# Autodesk Inventor assembly: Drivebase
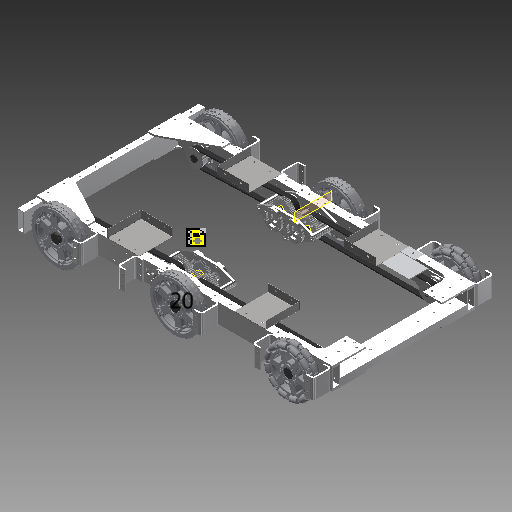
[picture p0: Inventor's stored thumbnail of the model, 512x512]
Saved by Autodesk Inventor 2019.4 (Build 234330000, 330)
## iProperties
Created: 2020-01-05
Part Number: Drivebase
Document SubType Name: Assembly
Designer: Mark
Mass: 13329.8 g
Surface Area: 29632.2 cm^2
Volume: 5059.07 cm^3
Density: 2.63483 g/cm^3
Author: Mark
## Documents named in this file (38)
- C:\Users\admin\Desktop\FRC 2020 Engineering\GitHub\7738-2020\CAD\Drivebase.iam
- C:\Users\admin\Desktop\FRC 2020 Engineering\GitHub\7738-2020\CAD\Main Extrusion.ipt
- C:\Users\admin\Desktop\FRC 2020 Engineering\GitHub\7738-2020\CAD\Back Extrusion.ipt
- C:\Users\admin\Desktop\FRC 2020 Engineering\GitHub\7738-2020\CAD\Bearing Block Assembly.iam
- C:\Users\admin\Desktop\FRC 2020 Engineering\GitHub\7738-2020\CAD\Gearbox\Drivebox.iam
- C:\Users\admin\Desktop\FRC 2020 Engineering\GitHub\7738-2020\CAD\End Extrusion.ipt
- C:\Users\admin\Desktop\FRC 2020 Engineering\GitHub\7738-2020\CAD\Gearbox\HTD 5M 30 20mm ID Keyed.ipt
- C:\Users\admin\Desktop\FRC 2020 Engineering\GitHub\7738-2020\CAD\Gearbox\30-30-870-HTD5M.ipt
- C:\Users\admin\Desktop\FRC 2020 Engineering\GitHub\7738-2020\CAD\Gearbox\30-30-750-HTD5M.ipt
- C:\Users\admin\Desktop\FRC 2020 Engineering\GitHub\7738-2020\CAD\Frontal Sheet Metal Support.ipt
- C:\Users\admin\Desktop\FRC 2020 Engineering\GitHub\7738-2020\CAD\Shaft-Secondary.ipt
- C:\Users\admin\Desktop\FRC 2020 Engineering\GitHub\7738-2020\CAD\Drivebase\Design Accelerator\Key Connection1.iam
- C:\Users\admin\Desktop\FRC 2020 Engineering\GitHub\7738-2020\CAD\Shaft-2.ipt
- C:\Users\admin\Desktop\FRC 2020 Engineering\GitHub\7738-2020\CAD\Back Brace.ipt
- C:\Users\admin\Desktop\FRC 2020 Engineering\GitHub\7738-2020\CAD\Back brace 2.ipt
- C:\Users\admin\Desktop\FRC 2020 Engineering\GitHub\7738-2020\CAD\Front Brace 2.ipt
- C:\Users\admin\Desktop\FRC 2020 Engineering\GitHub\7738-2020\CAD\Gearbox Support Thing.ipt
- C:\Users\admin\Desktop\FRC 2020 Engineering\GitHub\7738-2020\CAD\Main Extrusion_MIR.ipt
- C:\Users\admin\Desktop\FRC 2020 Engineering\GitHub\7738-2020\CAD\Bearing Block Assembly_MIR.iam
- C:\Users\admin\Desktop\FRC 2020 Engineering\GitHub\7738-2020\CAD\Gearbox\Drivebox_MIR.iam
- C:\Users\admin\Desktop\FRC 2020 Engineering\GitHub\7738-2020\CAD\Gearbox\HTD 5M 30 20mm ID Keyed_MIR.ipt
- C:\Users\admin\Desktop\FRC 2020 Engineering\GitHub\7738-2020\CAD\Gearbox\30-30-870-HTD5M_MIR.ipt
- C:\Users\admin\Desktop\FRC 2020 Engineering\GitHub\7738-2020\CAD\Gearbox\30-30-750-HTD5M_MIR.ipt
- C:\Users\admin\Desktop\FRC 2020 Engineering\GitHub\7738-2020\CAD\Frontal Sheet Metal Support_MIR.ipt
- C:\Users\admin\Desktop\FRC 2020 Engineering\GitHub\7738-2020\CAD\Shaft-Secondary_MIR.ipt
- C:\Users\admin\Desktop\FRC 2020 Engineering\GitHub\7738-2020\CAD\Drivebase\Design Accelerator\Key Connection1_MIR.iam
- C:\Users\admin\Desktop\FRC 2020 Engineering\GitHub\7738-2020\CAD\Shaft-Main_MIR.ipt
- C:\Users\admin\Desktop\FRC 2020 Engineering\GitHub\7738-2020\CAD\Shaft-2_MIR.ipt
- C:\Users\admin\Desktop\FRC 2020 Engineering\GitHub\7738-2020\CAD\Back Brace_MIR.ipt
- C:\Users\admin\Desktop\FRC 2020 Engineering\GitHub\7738-2020\CAD\Back brace 2_MIR.ipt
- C:\Users\admin\Desktop\FRC 2020 Engineering\GitHub\7738-2020\CAD\Gearbox Support Thing_MIR.ipt
- C:\Users\admin\Desktop\FRC 2020 Engineering\GitHub\7738-2020\CAD\Shaft-Main.ipt
- C:\Users\admin\Desktop\FRC 2020 Engineering\GitHub\7738-2020\CAD\6_Omni-Directional_Wheel_217-2585.ipt
- C:\Users\admin\Desktop\FRC 2020 Engineering\GitHub\7738-2020\CAD\6_Traction_Wheel_-_1_Wide_217-2589.ipt
- C:\Users\admin\Desktop\FRC 2020 Engineering\GitHub\7738-2020\CAD\6_Traction_Tire_-_0_5_Wide_217-2860.ipt
- C:\Users\admin\Desktop\FRC 2020 Engineering\GitHub\7738-2020\CAD\Sheet Metal Support.ipt
- C:\Users\admin\Desktop\FRC 2020 Engineering\GitHub\7738-2020\CAD\Sheet Metal Support_MIR.ipt
- C:\Users\admin\Desktop\FRC 2020 Engineering\GitHub\7738-2020\Battery Support.ipt
## Components (75 placed, 37 different names)
1. Main Extrusion:1 — Mate:1, Flush:1, Flush:2, Mate:2, Mate:3, Mate:4, Mate:5, Mate:6, Mate:7, Mate:8, Mate:9, Mate:10, Mate:11, Mate:12, Mate:13, Mate:14, Mate:15, Mate:16, Mate:17, Mate:18, Mate:19, Mate:27, Mate:30, Flush:3, Mate:31, Flush:4, Flush:5, Flush:6, Flush:7, Mate:42, Mate:43, Flush:8, Mate:49, Flush:11, Mate:61, Flush:14, Flush:15, Mate:63, Flush:18, Flush:19, Mate:64, Flush:20, Flush:21, Mate:65, Flush:22, Mate:124, Flush:43, Flush:44, Mate:163, Mate:164, Mate:165, Mate:168, Mate:176, Mate:177, Mate:178, Mate:179, Mate:180, Mate:181
2. Back Extrusion:1 — Mate:1, Flush:1, Flush:2, Mate:50, Mate:119, Flush:39, Flush:40
3. Bearing Block Assembly:1 [sub-assembly] — Mate:2, Mate:3, Mate:4, Mate:32, Mate:33
4. Bearing Block Assembly:2 [sub-assembly] — Mate:5, Mate:6, Mate:7, Mate:34, Mate:35
5. Bearing Block Assembly:3 [sub-assembly] — Mate:11, Mate:12, Mate:13, Mate:53, Mate:127
6. Bearing Block Assembly:4 [sub-assembly] — Mate:8, Mate:9, Mate:10, Mate:126
7. Bearing Block Assembly:5 [sub-assembly] — Mate:14, Mate:15, Mate:16, Mate:60, Flush:13
8. Bearing Block Assembly:6 [sub-assembly] — Mate:17, Mate:18, Mate:19, Mate:37, Mate:132, Mate:133
9. Drivebox:1 [sub-assembly] — Mate:27, Mate:31, Flush:4, Mate:40, Mate:121
10. End Extrusion:1 — Mate:30, Flush:3, Flush:5, Flush:46
11. HTD 5M 30 20mm ID Keyed:1 — Mate:32, Mate:33, Mate:39, Mate:41
12. HTD 5M 30 20mm ID Keyed:2 — Mate:34, Mate:35, Mate:36, Mate:38
13. 30-30-870-HTD5M:1 — Mate:36, Mate:37, Mate:38
14. 30-30-730-HTD5M:1 — Mate:39, Mate:40, Mate:41
15. Frontal Sheet Metal Support:1 — Flush:6, Flush:7, Mate:42, Mate:44
16. Frontal Sheet Metal Support:2 — Mate:43, Flush:8, Mate:44
17. Frontal Sheet Metal Support:5 — Mate:49, Flush:11, Mate:50
18. Shaft-Secondary:1 — Mate:53, Mate:127, Mate:140, Mate:141
19. Shaft-Secondary:2 — Mate:126, Mate:134, Mate:135
20. Key Connection:1 [sub-assembly]
21. Shaft-2:1 — Mate:60, Flush:13
22. Back Brace:1 — Mate:61, Flush:14, Flush:15
23. Back brace 2:1 — Mate:63, Flush:18, Flush:19
24. Front Brace 2:1 — Mate:64, Flush:20, Flush:21
25. Gearbox Support Thing:1 — Mate:65, Flush:22, Mate:121
26. Main Extrusion_MIR:1 — Mate:66, Mate:67, Mate:68, Mate:69, Mate:70, Mate:71, Mate:72, Mate:73, Mate:74, Mate:75, Mate:76, Mate:77, Mate:78, Mate:79, Mate:80, Mate:81, Mate:82, Mate:83, Flush:23, Mate:89, Mate:90, Mate:101, Flush:24, Flush:25, Flush:26, Mate:103, Flush:27, Mate:104, Flush:30, Flush:31, Mate:114, Flush:34, Flush:35, Mate:116, Flush:38, Mate:118, Mate:119, Flush:39, Flush:40, Mate:122, Mate:123, Flush:41, Flush:42, Mate:125, Flush:45, Flush:56, Mate:166, Mate:167, Mate:169, Flush:61, Mate:170, Mate:171, Mate:172, Mate:173, Mate:174, Mate:175, Mate:182, Mate:183
27. Bearing Block Assembly_MIR:1 [sub-assembly] — Mate:66, Mate:67, Mate:68, Mate:91, Mate:92
28. Bearing Block Assembly_MIR:2 [sub-assembly] — Mate:69, Mate:70, Mate:71, Mate:93, Mate:94
29. Bearing Block Assembly_MIR:3 [sub-assembly] — Mate:72, Mate:73, Mate:74, Mate:107, Mate:129
30. Bearing Block Assembly_MIR:4 [sub-assembly] — Mate:75, Mate:76, Mate:77, Mate:128, Mate:130
31. Bearing Block Assembly_MIR:5 [sub-assembly] — Mate:78, Mate:79, Mate:80, Flush:29, Mate:113
32. Bearing Block Assembly_MIR:6 [sub-assembly] — Mate:81, Mate:82, Mate:83, Mate:96, Mate:110, Mate:145
33. Drivebox_MIR:1 [sub-assembly] — Flush:23, Mate:89, Mate:90, Mate:99, Mate:131
34. HTD 5M 30 20mm ID Keyed_MIR:1 — Mate:91, Mate:92, Mate:98, Mate:100
35. HTD 5M 30 20mm ID Keyed_MIR:2 — Mate:93, Mate:94, Mate:95, Mate:97
36. 30-30-870-HTD5M_MIR:1 — Mate:95, Mate:96, Mate:97
37. 30-30-730-HTD5M_MIR:1 — Mate:98, Mate:99, Mate:100
38. Frontal Sheet Metal Support_MIR:1 — Mate:101, Flush:24, Flush:25, Mate:102
39. Frontal Sheet Metal Support_MIR:2 — Mate:102, Flush:26, Mate:103
40. Frontal Sheet Metal Support_MIR:3 — Flush:27, Mate:104, Mate:122
41. Shaft-Secondary_MIR:1 — Mate:107, Mate:129, Mate:142, Mate:143
42. Shaft-Secondary_MIR:2 — Mate:128, Mate:130, Mate:136, Mate:137
43. Key Connection1_MIR:1 [sub-assembly]
44. Shaft-Main_MIR:1 — Mate:110, Mate:144, Mate:145, Mate:146
45. Shaft-2_MIR:1 — Flush:29, Mate:113
46. Back Brace_MIR:1 — Flush:30, Flush:31, Mate:114
47. Back brace 2_MIR:1 — Flush:34, Flush:35, Mate:116
48. Gearbox Support Thing_MIR:1 — Flush:38, Mate:118, Mate:131
49. Front Brace 2:2 — Mate:123, Flush:41, Flush:42, Mate:184
50. Front Brace 2:3 — Mate:124, Flush:43, Flush:44
51. Front Brace 2:4 — Mate:125, Flush:45, Flush:46
52. Shaft-Main:1 — Mate:132, Mate:133, Mate:138, Mate:139
53. 6_Omni-Directional_Wheel_217-2585:1 — Mate:136, Mate:137
54. 6_Omni-Directional_Wheel_217-2585:2 — Mate:134, Mate:135
55. 6_Traction_Wheel_-_1_Wide_217-2589:1 — Mate:144, Mate:146, Mate:159, Mate:160, Mate:161
56. 6_Traction_Wheel_-_1_Wide_217-2589:2 — Mate:140, Mate:141, Mate:147, Mate:148, Mate:149, Mate:150
57. 6_Traction_Wheel_-_1_Wide_217-2589:3 — Mate:142, Mate:143, Mate:155, Mate:156, Mate:157
58. 6_Traction_Wheel_-_1_Wide_217-2589:4 — Mate:138, Mate:139, Mate:151, Mate:152, Mate:153
59. 6_Traction_Tire_-_0_5_Wide_217-2860:1 — Mate:147, Mate:148
60. 6_Traction_Tire_-_0_5_Wide_217-2860:2 — Mate:151, Mate:152, Mate:154
61. 6_Traction_Tire_-_0_5_Wide_217-2860:3 — Mate:155, Mate:156, Mate:158
62. 6_Traction_Tire_-_0_5_Wide_217-2860:4 — Mate:153, Mate:154
63. 6_Traction_Tire_-_0_5_Wide_217-2860:5 — Mate:159, Mate:160, Mate:162
64. 6_Traction_Tire_-_0_5_Wide_217-2860:6 — Mate:157, Mate:158
65. 6_Traction_Tire_-_0_5_Wide_217-2860:7 — Mate:149, Mate:150
66. 6_Traction_Tire_-_0_5_Wide_217-2860:8 — Mate:161, Mate:162
67. Sheet Metal Support:1 — Mate:163, Mate:164, Mate:165, Flush:58, Flush:60
68. Sheet Metal Support:3 — Flush:56, Flush:57, Flush:59, Mate:166, Mate:167
69. Sheet Metal Support_MIR:1 — Flush:58, Flush:59, Mate:168
70. Sheet Metal Support:4 — Mate:169, Flush:60, Flush:61
71. Frontal Sheet Metal Support_MIR:4 — Mate:170, Mate:171, Mate:175
72. Frontal Sheet Metal Support_MIR:5 — Mate:172, Mate:173, Mate:174
73. Frontal Sheet Metal Support_MIR:6 — Mate:176, Mate:177, Mate:181
74. Frontal Sheet Metal Support_MIR:7 — Mate:178, Mate:179, Mate:180
75. Battery Support:1 — Mate:182, Mate:183, Mate:184
## Relationships (190: Mate 148, Flush 42)
- Mate:1: Main Extrusion:1 ↔ Back Extrusion:1
- Flush:1: Main Extrusion:1 ↔ Back Extrusion:1
- Flush:2 (-60 mm): Main Extrusion:1 ↔ Back Extrusion:1
- Mate:2: Main Extrusion:1 ↔ Bearing Block Assembly:1
- Mate:3: Main Extrusion:1 ↔ Bearing Block Assembly:1
- Mate:4: Main Extrusion:1 ↔ Bearing Block Assembly:1
- Mate:5: Main Extrusion:1 ↔ Bearing Block Assembly:2
- Mate:6: Main Extrusion:1 ↔ Bearing Block Assembly:2
- Mate:7: Main Extrusion:1 ↔ Bearing Block Assembly:2
- Mate:8: Main Extrusion:1 ↔ Bearing Block Assembly:4
- Mate:9: Main Extrusion:1 ↔ Bearing Block Assembly:4
- Mate:10: Main Extrusion:1 ↔ Bearing Block Assembly:4
- Mate:11: Main Extrusion:1 ↔ Bearing Block Assembly:3
- Mate:12: Main Extrusion:1 ↔ Bearing Block Assembly:3
- Mate:13: Main Extrusion:1 ↔ Bearing Block Assembly:3
- Mate:14: Main Extrusion:1 ↔ Bearing Block Assembly:5
- Mate:15: Main Extrusion:1 ↔ Bearing Block Assembly:5
- Mate:16: Main Extrusion:1 ↔ Bearing Block Assembly:5
- Mate:17: Main Extrusion:1 ↔ Bearing Block Assembly:6
- Mate:18: Main Extrusion:1 ↔ Bearing Block Assembly:6
- Mate:19: Main Extrusion:1 ↔ Bearing Block Assembly:6
- Mate:27: Main Extrusion:1 ↔ Drivebox:1
- Mate:30: Main Extrusion:1 ↔ End Extrusion:1
- Flush:3: Main Extrusion:1 ↔ End Extrusion:1
- Mate:31: Main Extrusion:1 ↔ Drivebox:1
- Flush:4: Main Extrusion:1 ↔ Drivebox:1
- Mate:32: Bearing Block Assembly:1 ↔ HTD 5M 30 20mm ID Keyed:1
- Mate:33 (3 mm): Bearing Block Assembly:1 ↔ HTD 5M 30 20mm ID Keyed:1
- Flush:5: Main Extrusion:1 ↔ End Extrusion:1
- Mate:34: Bearing Block Assembly:2 ↔ HTD 5M 30 20mm ID Keyed:2
- Mate:35 (3 mm): Bearing Block Assembly:2 ↔ HTD 5M 30 20mm ID Keyed:2
- Mate:36: HTD 5M 30 20mm ID Keyed:2 ↔ 30-30-870-HTD5M:1
- Mate:37: Bearing Block Assembly:6 ↔ 30-30-870-HTD5M:1
- Mate:38 (0.5 mm): HTD 5M 30 20mm ID Keyed:2 ↔ 30-30-870-HTD5M:1
- Mate:39: HTD 5M 30 20mm ID Keyed:1 ↔ 30-30-730-HTD5M:1
- Mate:40: Drivebox:1 ↔ 30-30-730-HTD5M:1
- Mate:41 (0.5 mm): HTD 5M 30 20mm ID Keyed:1 ↔ 30-30-730-HTD5M:1
- Flush:6: Main Extrusion:1 ↔ Frontal Sheet Metal Support:1
- Flush:7: Main Extrusion:1 ↔ Frontal Sheet Metal Support:1
- Mate:42: Main Extrusion:1 ↔ Frontal Sheet Metal Support:1
- Mate:43: Main Extrusion:1 ↔ Frontal Sheet Metal Support:2
- Flush:8: Main Extrusion:1 ↔ Frontal Sheet Metal Support:2
- Mate:44 (143 mm): Frontal Sheet Metal Support:1 ↔ Frontal Sheet Metal Support:2
- Mate:49: Main Extrusion:1 ↔ Frontal Sheet Metal Support:5
- Flush:11: Main Extrusion:1 ↔ Frontal Sheet Metal Support:5
- Mate:50 (173 mm): Back Extrusion:1 ↔ Frontal Sheet Metal Support:5
- Mate:53: Bearing Block Assembly:3 ↔ Shaft-Secondary:1
- Mate:60: Bearing Block Assembly:5 ↔ Shaft-2:1
- Flush:13 (-0.2 mm): Bearing Block Assembly:5 ↔ Shaft-2:1
- Mate:61: Main Extrusion:1 ↔ Back Brace:1
- Flush:14: Main Extrusion:1 ↔ Back Brace:1
- Flush:15 (-20 mm): Main Extrusion:1 ↔ Back Brace:1
- Mate:63: Main Extrusion:1 ↔ Back brace 2:1
- Flush:18: Main Extrusion:1 ↔ Back brace 2:1
- Flush:19 (-20 mm): Main Extrusion:1 ↔ Back brace 2:1
- Mate:64: Main Extrusion:1 ↔ Front Brace 2:1
- Flush:20: Main Extrusion:1 ↔ Front Brace 2:1
- Flush:21: Main Extrusion:1 ↔ Front Brace 2:1
- Mate:65: Main Extrusion:1 ↔ Gearbox Support Thing:1
- Flush:22: Main Extrusion:1 ↔ Gearbox Support Thing:1
- Mate:66: Main Extrusion_MIR:1 ↔ Bearing Block Assembly_MIR:1
- Mate:67: Main Extrusion_MIR:1 ↔ Bearing Block Assembly_MIR:1
- Mate:68: Main Extrusion_MIR:1 ↔ Bearing Block Assembly_MIR:1
- Mate:69: Main Extrusion_MIR:1 ↔ Bearing Block Assembly_MIR:2
- Mate:70: Main Extrusion_MIR:1 ↔ Bearing Block Assembly_MIR:2
- Mate:71: Main Extrusion_MIR:1 ↔ Bearing Block Assembly_MIR:2
- Mate:72: Main Extrusion_MIR:1 ↔ Bearing Block Assembly_MIR:3
- Mate:73: Main Extrusion_MIR:1 ↔ Bearing Block Assembly_MIR:3
- Mate:74: Main Extrusion_MIR:1 ↔ Bearing Block Assembly_MIR:3
- Mate:75: Main Extrusion_MIR:1 ↔ Bearing Block Assembly_MIR:4
- Mate:76: Main Extrusion_MIR:1 ↔ Bearing Block Assembly_MIR:4
- Mate:77: Main Extrusion_MIR:1 ↔ Bearing Block Assembly_MIR:4
- Mate:78: Main Extrusion_MIR:1 ↔ Bearing Block Assembly_MIR:5
- Mate:79: Main Extrusion_MIR:1 ↔ Bearing Block Assembly_MIR:5
- Mate:80: Main Extrusion_MIR:1 ↔ Bearing Block Assembly_MIR:5
- Mate:81: Main Extrusion_MIR:1 ↔ Bearing Block Assembly_MIR:6
- Mate:82: Main Extrusion_MIR:1 ↔ Bearing Block Assembly_MIR:6
- Mate:83: Main Extrusion_MIR:1 ↔ Bearing Block Assembly_MIR:6
- Flush:23: Main Extrusion_MIR:1 ↔ Drivebox_MIR:1
- Mate:89: Main Extrusion_MIR:1 ↔ Drivebox_MIR:1
- Mate:90: Main Extrusion_MIR:1 ↔ Drivebox_MIR:1
- Mate:91 (3 mm): Bearing Block Assembly_MIR:1 ↔ HTD 5M 30 20mm ID Keyed_MIR:1
- Mate:92: Bearing Block Assembly_MIR:1 ↔ HTD 5M 30 20mm ID Keyed_MIR:1
- Mate:93 (3 mm): Bearing Block Assembly_MIR:2 ↔ HTD 5M 30 20mm ID Keyed_MIR:2
- Mate:94: Bearing Block Assembly_MIR:2 ↔ HTD 5M 30 20mm ID Keyed_MIR:2
- Mate:95 (0.5 mm): HTD 5M 30 20mm ID Keyed_MIR:2 ↔ 30-30-870-HTD5M_MIR:1
- Mate:96: Bearing Block Assembly_MIR:6 ↔ 30-30-870-HTD5M_MIR:1
- Mate:97: HTD 5M 30 20mm ID Keyed_MIR:2 ↔ 30-30-870-HTD5M_MIR:1
- Mate:98 (0.5 mm): HTD 5M 30 20mm ID Keyed_MIR:1 ↔ 30-30-730-HTD5M_MIR:1
- Mate:99: Drivebox_MIR:1 ↔ 30-30-730-HTD5M_MIR:1
- Mate:100: HTD 5M 30 20mm ID Keyed_MIR:1 ↔ 30-30-730-HTD5M_MIR:1
- Mate:101: Main Extrusion_MIR:1 ↔ Frontal Sheet Metal Support_MIR:1
- Flush:24: Main Extrusion_MIR:1 ↔ Frontal Sheet Metal Support_MIR:1
- Flush:25: Main Extrusion_MIR:1 ↔ Frontal Sheet Metal Support_MIR:1
- Mate:102 (140 mm): Frontal Sheet Metal Support_MIR:1 ↔ Frontal Sheet Metal Support_MIR:2
- Flush:26: Main Extrusion_MIR:1 ↔ Frontal Sheet Metal Support_MIR:2
- Mate:103: Main Extrusion_MIR:1 ↔ Frontal Sheet Metal Support_MIR:2
- Flush:27: Main Extrusion_MIR:1 ↔ Frontal Sheet Metal Support_MIR:3
- Mate:104: Main Extrusion_MIR:1 ↔ Frontal Sheet Metal Support_MIR:3
- Mate:107: Bearing Block Assembly_MIR:3 ↔ Shaft-Secondary_MIR:1
- Mate:110 (6 mm): Bearing Block Assembly_MIR:6 ↔ Shaft-Main_MIR:1
- Flush:29 (-0.2 mm): Bearing Block Assembly_MIR:5 ↔ Shaft-2_MIR:1
- Mate:113: Bearing Block Assembly_MIR:5 ↔ Shaft-2_MIR:1
- Flush:30 (-20 mm): Main Extrusion_MIR:1 ↔ Back Brace_MIR:1
- Flush:31: Main Extrusion_MIR:1 ↔ Back Brace_MIR:1
- Mate:114: Main Extrusion_MIR:1 ↔ Back Brace_MIR:1
- Flush:34 (-20 mm): Main Extrusion_MIR:1 ↔ Back brace 2_MIR:1
- Flush:35: Main Extrusion_MIR:1 ↔ Back brace 2_MIR:1
- Mate:116: Main Extrusion_MIR:1 ↔ Back brace 2_MIR:1
- Flush:38: Main Extrusion_MIR:1 ↔ Gearbox Support Thing_MIR:1
- Mate:118: Main Extrusion_MIR:1 ↔ Gearbox Support Thing_MIR:1
- Mate:119: Back Extrusion:1 ↔ Main Extrusion_MIR:1
- Flush:39: Back Extrusion:1 ↔ Main Extrusion_MIR:1
- Flush:40 (60 mm): Back Extrusion:1 ↔ Main Extrusion_MIR:1
- Mate:121: Drivebox:1 ↔ Gearbox Support Thing:1
- Mate:122: Main Extrusion_MIR:1 ↔ Frontal Sheet Metal Support_MIR:3
- Mate:123: Main Extrusion_MIR:1 ↔ Front Brace 2:2
- Flush:41: Main Extrusion_MIR:1 ↔ Front Brace 2:2
- Flush:42: Main Extrusion_MIR:1 ↔ Front Brace 2:2
- Mate:124: Main Extrusion:1 ↔ Front Brace 2:3
- Flush:43: Main Extrusion:1 ↔ Front Brace 2:3
- Flush:44: Main Extrusion:1 ↔ Front Brace 2:3
- Mate:125: Main Extrusion_MIR:1 ↔ Front Brace 2:4
- Flush:45: Main Extrusion_MIR:1 ↔ Front Brace 2:4
- Flush:46: End Extrusion:1 ↔ Front Brace 2:4
- Mate:126 (6 mm): Bearing Block Assembly:4 ↔ Shaft-Secondary:2
- Mate:127 (6 mm): Bearing Block Assembly:3 ↔ Shaft-Secondary:1
- Mate:128 (6 mm): Bearing Block Assembly_MIR:4 ↔ Shaft-Secondary_MIR:2
- Mate:129 (6 mm): Bearing Block Assembly_MIR:3 ↔ Shaft-Secondary_MIR:1
- Mate:130: Bearing Block Assembly_MIR:4 ↔ Shaft-Secondary_MIR:2
- Mate:131: Drivebox_MIR:1 ↔ Gearbox Support Thing_MIR:1
- Mate:132: Bearing Block Assembly:6 ↔ Shaft-Main:1
- Mate:133 (6 mm): Bearing Block Assembly:6 ↔ Shaft-Main:1
- Mate:134: Shaft-Secondary:2 ↔ 6_Omni-Directional_Wheel_217-2585:2
- Mate:135: Shaft-Secondary:2 ↔ 6_Omni-Directional_Wheel_217-2585:2
- Mate:136: Shaft-Secondary_MIR:2 ↔ 6_Omni-Directional_Wheel_217-2585:1
- Mate:137: Shaft-Secondary_MIR:2 ↔ 6_Omni-Directional_Wheel_217-2585:1
- Mate:138: Shaft-Main:1 ↔ 6_Traction_Wheel_-_1_Wide_217-2589:4
- Mate:139: Shaft-Main:1 ↔ 6_Traction_Wheel_-_1_Wide_217-2589:4
- Mate:140: Shaft-Secondary:1 ↔ 6_Traction_Wheel_-_1_Wide_217-2589:2
- Mate:141: Shaft-Secondary:1 ↔ 6_Traction_Wheel_-_1_Wide_217-2589:2
- Mate:142: Shaft-Secondary_MIR:1 ↔ 6_Traction_Wheel_-_1_Wide_217-2589:3
- Mate:143: Shaft-Secondary_MIR:1 ↔ 6_Traction_Wheel_-_1_Wide_217-2589:3
- Mate:144: Shaft-Main_MIR:1 ↔ 6_Traction_Wheel_-_1_Wide_217-2589:1
- Mate:145: Bearing Block Assembly_MIR:6 ↔ Shaft-Main_MIR:1
- Mate:146: Shaft-Main_MIR:1 ↔ 6_Traction_Wheel_-_1_Wide_217-2589:1
- Mate:147: 6_Traction_Wheel_-_1_Wide_217-2589:2 ↔ 6_Traction_Tire_-_0_5_Wide_217-2860:1
- Mate:148: 6_Traction_Wheel_-_1_Wide_217-2589:2 ↔ 6_Traction_Tire_-_0_5_Wide_217-2860:1
- Mate:149: 6_Traction_Wheel_-_1_Wide_217-2589:2 ↔ 6_Traction_Tire_-_0_5_Wide_217-2860:7
- Mate:150: 6_Traction_Wheel_-_1_Wide_217-2589:2 ↔ 6_Traction_Tire_-_0_5_Wide_217-2860:7
- Mate:151: 6_Traction_Wheel_-_1_Wide_217-2589:4 ↔ 6_Traction_Tire_-_0_5_Wide_217-2860:2
- Mate:152: 6_Traction_Wheel_-_1_Wide_217-2589:4 ↔ 6_Traction_Tire_-_0_5_Wide_217-2860:2
- Mate:153: 6_Traction_Wheel_-_1_Wide_217-2589:4 ↔ 6_Traction_Tire_-_0_5_Wide_217-2860:4
- Mate:154: 6_Traction_Tire_-_0_5_Wide_217-2860:2 ↔ 6_Traction_Tire_-_0_5_Wide_217-2860:4
- Mate:155: 6_Traction_Wheel_-_1_Wide_217-2589:3 ↔ 6_Traction_Tire_-_0_5_Wide_217-2860:3
- Mate:156: 6_Traction_Wheel_-_1_Wide_217-2589:3 ↔ 6_Traction_Tire_-_0_5_Wide_217-2860:3
- Mate:157: 6_Traction_Wheel_-_1_Wide_217-2589:3 ↔ 6_Traction_Tire_-_0_5_Wide_217-2860:6
- Mate:158: 6_Traction_Tire_-_0_5_Wide_217-2860:3 ↔ 6_Traction_Tire_-_0_5_Wide_217-2860:6
- Mate:159: 6_Traction_Wheel_-_1_Wide_217-2589:1 ↔ 6_Traction_Tire_-_0_5_Wide_217-2860:5
- Mate:160: 6_Traction_Wheel_-_1_Wide_217-2589:1 ↔ 6_Traction_Tire_-_0_5_Wide_217-2860:5
- Mate:161: 6_Traction_Wheel_-_1_Wide_217-2589:1 ↔ 6_Traction_Tire_-_0_5_Wide_217-2860:8
- Mate:162: 6_Traction_Tire_-_0_5_Wide_217-2860:5 ↔ 6_Traction_Tire_-_0_5_Wide_217-2860:8
- Mate:163: Main Extrusion:1 ↔ Sheet Metal Support:1
- Mate:164: Main Extrusion:1 ↔ Sheet Metal Support:1
- Mate:165: Main Extrusion:1 ↔ Sheet Metal Support:1
- Flush:56: Main Extrusion_MIR:1 ↔ Sheet Metal Support:3
- Flush:57 (150 mm): Sheet Metal Support:3
- Flush:58: Sheet Metal Support:1 ↔ Sheet Metal Support_MIR:1
- Flush:59: Sheet Metal Support:3 ↔ Sheet Metal Support_MIR:1
- Mate:166: Main Extrusion_MIR:1 ↔ Sheet Metal Support:3
- Mate:167: Main Extrusion_MIR:1 ↔ Sheet Metal Support:3
- Mate:168: Main Extrusion:1 ↔ Sheet Metal Support_MIR:1
- Mate:169: Main Extrusion_MIR:1 ↔ Sheet Metal Support:4
- Flush:60: Sheet Metal Support:1 ↔ Sheet Metal Support:4
- Flush:61: Main Extrusion_MIR:1 ↔ Sheet Metal Support:4
- Mate:170: Main Extrusion_MIR:1 ↔ Frontal Sheet Metal Support_MIR:4
- Mate:171: Main Extrusion_MIR:1 ↔ Frontal Sheet Metal Support_MIR:4
- Mate:172: Main Extrusion_MIR:1 ↔ Frontal Sheet Metal Support_MIR:5
- Mate:173: Main Extrusion_MIR:1 ↔ Frontal Sheet Metal Support_MIR:5
- Mate:174: Main Extrusion_MIR:1 ↔ Frontal Sheet Metal Support_MIR:5
- Mate:175: Main Extrusion_MIR:1 ↔ Frontal Sheet Metal Support_MIR:4
- Mate:176: Main Extrusion:1 ↔ Frontal Sheet Metal Support_MIR:6
- Mate:177: Main Extrusion:1 ↔ Frontal Sheet Metal Support_MIR:6
- Mate:178: Main Extrusion:1 ↔ Frontal Sheet Metal Support_MIR:7
- Mate:179: Main Extrusion:1 ↔ Frontal Sheet Metal Support_MIR:7
- Mate:180: Main Extrusion:1 ↔ Frontal Sheet Metal Support_MIR:7
- Mate:181: Main Extrusion:1 ↔ Frontal Sheet Metal Support_MIR:6
- Mate:182: Main Extrusion_MIR:1 ↔ Battery Support:1
- Mate:183: Main Extrusion_MIR:1 ↔ Battery Support:1
- Mate:184: Front Brace 2:2 ↔ Battery Support:1
